# Autodesk Inventor assembly: central_gear
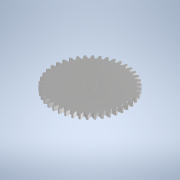
[picture p0: Inventor's stored thumbnail of the model, 180x180]
Saved by Autodesk Inventor 2020.2 (Build 242310000, 310)
## iProperties
Created: 2020-09-17
Part Number: central_gear
Document SubType Name: Assembly
Designer: mazzo
Author: mazzo
## Documents named in this file (2)
- D:\Documenti\università\Progetto Meccanica dei Robot\assembled in urdf\central_gear.iam
- D:\Documenti\università\Progetto Meccanica dei Robot\meccanica\parti autodesk\V5\Ingranaggio cilindrico centrale.ipt
## Components (1 placed, 1 different names)
1. Ingranaggio cilindrico2:1 — Coincidente:1, Coincidente:2
## Relationships (2: Mate 2)
- Coincidente:1 [Mate]: Ingranaggio cilindrico2:1
- Coincidente:2 [Mate]: Ingranaggio cilindrico2:1
